# Autodesk Inventor assembly: radio_assembly
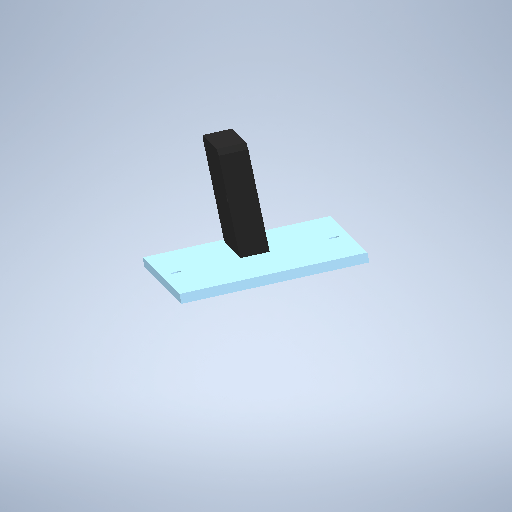
[picture p0: Inventor's stored thumbnail of the model, 512x512]
Saved by Autodesk Inventor 2025.3 (Build 293356000, 356)
## iProperties
Created: 2026-02-19
Part Number: radio_assembly
Document SubType Name: Assembly
Designer: m263126
Author: m263126
## Documents named in this file (3)
- C:\Users\m263126\Documents\EW401 Capstone\CAD Files\Brackets\radio_assembly.iam
- C:\Users\m263126\Documents\EW401 Capstone\CAD Files\Brackets\4x2_bracket.ipt
- C:\Users\m263126\Documents\EW401 Capstone\CAD Files\Sensors\Radio Mount.ipt
## Components (2 placed, 2 different names)
1. 4x2_bracket:1 — Mate:1, Mate:2, Flush:1, Flush:2
2. Radio Mount:1 — Mate:1, Mate:2, Flush:1, Flush:2
## Relationships (4: Mate 2, Flush 2)
- Mate:1: 4x2_bracket:1 ↔ Radio Mount:1
- Mate:2: 4x2_bracket:1 ↔ Radio Mount:1
- Flush:1 (50.8 mm): 4x2_bracket:1 ↔ Radio Mount:1
- Flush:2 (-25.4 mm): 4x2_bracket:1 ↔ Radio Mount:1
